# Autodesk Inventor assembly: Hand
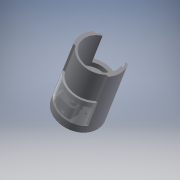
[picture p0: Inventor's stored thumbnail of the model, 180x180]
Saved by Autodesk Inventor 2016 (Build 200138000, 138)
## iProperties
Created: 2016-11-12
Part Number: Hand
Material: 一般
Document SubType Name: Assembly
Designer: Daisuke
Author: Daisuke
## Documents named in this file (6)
- C:\Users\Daisuke\Documents\GitHub\CAD\Hand\ver1\Hand.iam
- C:\Users\Daisuke\Documents\GitHub\CAD\Hand\ver1\insideHand.iam
- C:\Users\Daisuke\Documents\GitHub\CAD\Hand\ver1\outsideHand.iam
- C:\Users\Daisuke\Documents\GitHub\CAD\Hand\ver1\Servo.iam
- C:\Users\Daisuke\Documents\GitHub\CAD\Hand\ver1\ServoArm.ipt
- C:\Users\Daisuke\Documents\GitHub\CAD\Hand\ver1\Servo.ipt
## Components (5 placed, 4 different names)
1. insideHand:1 [sub-assembly] — 挿入:3
2. outsideHand:1 [sub-assembly] — 挿入:1, 挿入:2, 挿入:3, 挿入:4, 挿入:5
3. Servo:1 [sub-assembly] — 挿入:1, 挿入:2
4. ServoArm:1 — 挿入:4, 挿入:5, 挿入:6
5. Servo:2 — 挿入:6
## Relationships (6: Insert 6)
- 挿入:1 [Insert]: outsideHand:1 ↔ Servo:1
- 挿入:2 [Insert]: outsideHand:1 ↔ Servo:1
- 挿入:3 [Insert]: insideHand:1 ↔ outsideHand:1
- 挿入:4 [Insert]: outsideHand:1 ↔ ServoArm:1
- 挿入:5 [Insert]: outsideHand:1 ↔ ServoArm:1
- 挿入:6 [Insert] (0.5 mm): ServoArm:1 ↔ Servo:2
